# Autodesk Inventor assembly: final_MK4
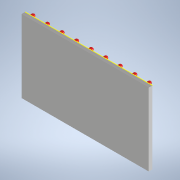
[picture p0: Inventor's stored thumbnail of the model, 180x180]
Saved by Autodesk Inventor 2020 (Build 240168000, 168)
## iProperties
Created: 2020-01-23
Part Number: final_MK4
Document SubType Name: Assembly
Designer: sl65b
Author: sl65b
## Documents named in this file (3)
- C:\Users\sl65b\Desktop\Laboratory\MODEL\material_MK4\final_MK4.iam
- C:\Users\sl65b\Desktop\Laboratory\MODEL\material_MK4\soft_all.ipt
- C:\Users\sl65b\Desktop\Laboratory\MODEL\material_MK4\hard_all.ipt
## Components (2 placed, 2 different names)
1. soft_all:1 — Rigid:1
2. hard_all:1 — Rigid:1
## Relationships (1: WeldJoint 1)
- Rigid:1 [WeldJoint] (0.01 mm): soft_all:1 ↔ hard_all:1
